# Autodesk Inventor assembly: Escritorio
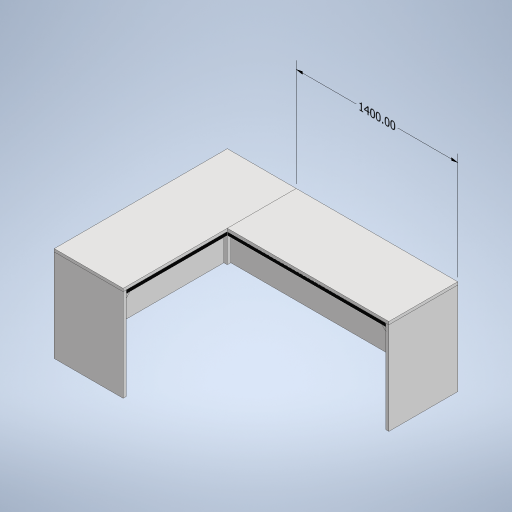
[picture p0: Inventor's stored thumbnail of the model, 512x512]
Saved by Autodesk Inventor 2024 (Build 280153000, 153)
## iProperties
Created: 2023-07-02
Part Number: Escritorio
Document SubType Name: Assembly
Designer: sergi
Author: sergi
## Documents named in this file (17)
- C:\Users\sergi\OneDrive\Escritorio\Piso\Escritorio Piso\Escritorio.iam
- C:\Users\sergi\OneDrive\Escritorio\Piso\Escritorio Piso\Tablero 2.ipt
- C:\Users\sergi\OneDrive\Escritorio\Piso\Escritorio Piso\Lateral1.ipt
- C:\Users\sergi\OneDrive\Escritorio\Piso\Escritorio Piso\Lateral2.ipt
- C:\Users\sergi\OneDrive\Escritorio\Piso\Escritorio Piso\Barra1.ipt
- C:\Users\sergi\OneDrive\Escritorio\Piso\Escritorio Piso\TableroVertical1.ipt
- C:\Users\sergi\OneDrive\Escritorio\Piso\Escritorio Piso\TableroVertical2.ipt
- C:\Users\sergi\OneDrive\Escritorio\Piso\Escritorio Piso\Pata1.ipt
- C:\Users\sergi\OneDrive\Documentos\Tablero Superior Izquierdo.ipt
- C:\Users\sergi\OneDrive\Documentos\Union.ipt
- C:\Users\sergi\OneDrive\Escritorio\Piso\Escritorio Piso\Union.ipt
- C:\Users\sergi\OneDrive\Escritorio\Piso\Escritorio Piso\BarraMarco1.1.ipt
- C:\Users\sergi\OneDrive\Escritorio\Piso\Escritorio Piso\BarraMarco1.2.ipt
- C:\Users\sergi\OneDrive\Escritorio\Piso\Escritorio Piso\BarraMarco2.1.ipt
- C:\Users\sergi\OneDrive\Escritorio\Piso\Escritorio Piso\BarraMarco2.2.ipt
- C:\Users\sergi\OneDrive\Escritorio\Piso\Escritorio Piso\Inclinada3.ipt
- C:\Users\sergi\OneDrive\Escritorio\Piso\Escritorio Piso\Inclinada4.ipt
## Components (26 placed, 15 different names)
1. Tablero 2:1 — Coincidencia:3, Nivelación:5, Nivelación:6, Coincidencia:18, Nivelación:9, Nivelación:14, Coincidencia:52
2. Lateral1:1 — Coincidencia:16, Nivelación:13, Nivelación:15, Coincidencia:20, Nivelación:16, Coincidencia:22, Coincidencia:23, Coincidencia:24, Coincidencia:40, Coincidencia:45
3. Lateral2:1 — Coincidencia:3, Nivelación:5, Nivelación:6, Coincidencia:17, Coincidencia:34, Coincidencia:37, Coincidencia:38, Coincidencia:39, Coincidencia:44
4. Barra1:1 — Coincidencia:19, Nivelación:10, Nivelación:11, Coincidencia:21, Coincidencia:25, Coincidencia:26, Coincidencia:27, Nivelación:17, Coincidencia:35, Nivelación:18, Coincidencia:36
5. TableroVertical1:1 — Coincidencia:16
6. TableroVertical2:1 — Coincidencia:17, Coincidencia:18, Nivelación:9, Nivelación:29, Nivelación:30
7. Pata1:1 — Coincidencia:19, Nivelación:10, Nivelación:11
8. Tablero Superior Izquierdo:1 — Nivelación:13, Nivelación:14, Nivelación:15, Nivelación:17, Coincidencia:41, Nivelación:21, Coincidencia:43, Coincidencia:56, Coincidencia:57, Nivelación:31
9. Union:1 — Coincidencia:20, Coincidencia:21, Nivelación:16, Coincidencia:28
10. Union:2 — Coincidencia:24, Coincidencia:27, Coincidencia:28, Coincidencia:29
11. Union:3 — Coincidencia:23, Coincidencia:26, Coincidencia:29, Coincidencia:30
12. Union:4 — Coincidencia:22, Coincidencia:25, Coincidencia:30, Coincidencia:47
13. Union:5 — Coincidencia:34, Coincidencia:35, Nivelación:18, Nivelación:22
14. Union:6 — Nivelación:19, Coincidencia:37
15. Union:7 — Nivelación:19, Nivelación:20, Coincidencia:38
16. Union:8 — Nivelación:20, Coincidencia:36, Coincidencia:39, Coincidencia:49, Nivelación:23
17. BarraMarco1.1:1 — Coincidencia:40, Coincidencia:41, Nivelación:21, Coincidencia:46
18. BarraMarco1.2:1 — Coincidencia:43, Coincidencia:44, Nivelación:22, Coincidencia:48, Coincidencia:51, Nivelación:24, Nivelación:25
19. BarraMarco2.1:1 — Coincidencia:48, Coincidencia:49, Nivelación:23, Coincidencia:53
20. BarraMarco2.2:1 — Coincidencia:45, Coincidencia:46, Coincidencia:47, Coincidencia:55, Nivelación:27
21. BarraMarco1.2:2 — Nivelación:26, Coincidencia:52, Coincidencia:53
22. BarraMarco2.1:2 — Coincidencia:51, Nivelación:24, Nivelación:25, Nivelación:26
23. BarraMarco1.1:2 — Coincidencia:55, Nivelación:27, Coincidencia:56, Nivelación:28
24. BarraMarco2.2:2 — Nivelación:28, Coincidencia:57
25. Inclinada3:1 — Nivelación:29, Nivelación:30, Nivelación:31, Coincidencia:59, Coincidencia:60
26. Inclinada4:1 — Coincidencia:59, Coincidencia:60
## Relationships (68: Mate 44, Flush 24)
- Coincidencia:3 [Mate]: Tablero 2:1 ↔ Lateral2:1
- Nivelación:5 [Flush]: Tablero 2:1 ↔ Lateral2:1
- Nivelación:6 [Flush]: Tablero 2:1 ↔ Lateral2:1
- Coincidencia:16 [Mate]: Lateral1:1 ↔ TableroVertical1:1
- Coincidencia:17 [Mate]: Lateral2:1 ↔ TableroVertical2:1
- Coincidencia:18 [Mate] (500 mm): Tablero 2:1 ↔ TableroVertical2:1
- Nivelación:9 [Flush]: Tablero 2:1 ↔ TableroVertical2:1
- Coincidencia:19 [Mate]: Barra1:1 ↔ Pata1:1
- Nivelación:10 [Flush]: Barra1:1 ↔ Pata1:1
- Nivelación:11 [Flush]: Barra1:1 ↔ Pata1:1
- Nivelación:13 [Flush]: Lateral1:1 ↔ Tablero Superior Izquierdo:1
- Nivelación:14 [Flush]: Tablero 2:1 ↔ Tablero Superior Izquierdo:1
- Nivelación:15 [Flush]: Lateral1:1 ↔ Tablero Superior Izquierdo:1
- Coincidencia:20 [Mate]: Lateral1:1 ↔ Union:1
- Coincidencia:21 [Mate]: Barra1:1 ↔ Union:1
- Nivelación:16 [Flush]: Lateral1:1 ↔ Union:1
- Coincidencia:22 [Mate]: Lateral1:1 ↔ Union:4
- Coincidencia:23 [Mate]: Lateral1:1 ↔ Union:3
- Coincidencia:24 [Mate]: Lateral1:1 ↔ Union:2
- Coincidencia:25 [Mate]: Barra1:1 ↔ Union:4
- Coincidencia:26 [Mate]: Barra1:1 ↔ Union:3
- Coincidencia:27 [Mate]: Barra1:1 ↔ Union:2
- Coincidencia:28 [Mate] (153.6667 mm): Union:1 ↔ Union:2
- Coincidencia:29 [Mate] (153.667 mm): Union:2 ↔ Union:3
- Coincidencia:30 [Mate] (153.667 mm): Union:3 ↔ Union:4
- Nivelación:17 [Flush]: Barra1:1 ↔ Tablero Superior Izquierdo:1
- [Mate] (153.6667 mm): Union:5 ↔ Union:6
- [Mate] (153.667 mm): Union:6 ↔ Union:7
- [Mate] (153.667 mm): Union:7 ↔ Union:8
- Coincidencia:34 [Mate]: Lateral2:1 ↔ Union:5
- Coincidencia:35 [Mate]: Barra1:1 ↔ Union:5
- Nivelación:18 [Flush]: Barra1:1 ↔ Union:5
- Nivelación:19 [Flush]: Union:6 ↔ Union:7
- Nivelación:20 [Flush]: Union:7 ↔ Union:8
- Coincidencia:36 [Mate]: Barra1:1 ↔ Union:8
- Coincidencia:37 [Mate]: Lateral2:1 ↔ Union:6
- Coincidencia:38 [Mate]: Lateral2:1 ↔ Union:7
- Coincidencia:39 [Mate]: Lateral2:1 ↔ Union:8
- Coincidencia:40 [Mate]: Lateral1:1 ↔ BarraMarco1.1:1
- Coincidencia:41 [Mate]: Tablero Superior Izquierdo:1 ↔ BarraMarco1.1:1
- Nivelación:21 [Flush] (30 mm): Tablero Superior Izquierdo:1 ↔ BarraMarco1.1:1
- Coincidencia:43 [Mate]: Tablero Superior Izquierdo:1 ↔ BarraMarco1.2:1
- Coincidencia:44 [Mate]: Lateral2:1 ↔ BarraMarco1.2:1
- Nivelación:22 [Flush]: Union:5 ↔ BarraMarco1.2:1
- Coincidencia:45 [Mate]: Lateral1:1 ↔ BarraMarco2.2:1
- Coincidencia:46 [Mate]: BarraMarco1.1:1 ↔ BarraMarco2.2:1
- Coincidencia:47 [Mate]: Union:4 ↔ BarraMarco2.2:1
- Coincidencia:48 [Mate]: BarraMarco1.2:1 ↔ BarraMarco2.1:1
- Coincidencia:49 [Mate]: Union:8 ↔ BarraMarco2.1:1
- Nivelación:23 [Flush]: Union:8 ↔ BarraMarco2.1:1
- [Mate]: BarraMarco1.2:2 ↔ BarraMarco2.1:2
- Coincidencia:51 [Mate]: BarraMarco1.2:1 ↔ BarraMarco2.1:2
- Nivelación:24 [Flush]: BarraMarco1.2:1 ↔ BarraMarco2.1:2
- Nivelación:25 [Flush]: BarraMarco1.2:1 ↔ BarraMarco2.1:2
- Nivelación:26 [Flush]: BarraMarco1.2:2 ↔ BarraMarco2.1:2
- Coincidencia:52 [Mate]: Tablero 2:1 ↔ BarraMarco1.2:2
- Coincidencia:53 [Mate]: BarraMarco2.1:1 ↔ BarraMarco1.2:2
- [Mate]: BarraMarco1.1:2 ↔ BarraMarco2.2:2
- Coincidencia:55 [Mate]: BarraMarco2.2:1 ↔ BarraMarco1.1:2
- Nivelación:27 [Flush]: BarraMarco2.2:1 ↔ BarraMarco1.1:2
- Coincidencia:56 [Mate]: Tablero Superior Izquierdo:1 ↔ BarraMarco1.1:2
- Nivelación:28 [Flush]: BarraMarco1.1:2 ↔ BarraMarco2.2:2
- Coincidencia:57 [Mate]: Tablero Superior Izquierdo:1 ↔ BarraMarco2.2:2
- Nivelación:29 [Flush]: TableroVertical2:1 ↔ Inclinada3:1
- Nivelación:30 [Flush]: TableroVertical2:1 ↔ Inclinada3:1
- Nivelación:31 [Flush]: Tablero Superior Izquierdo:1 ↔ Inclinada3:1
- Coincidencia:59 [Mate]: Inclinada3:1 ↔ Inclinada4:1
- Coincidencia:60 [Mate]: Inclinada3:1 ↔ Inclinada4:1
## Named parameters: d55_d51 = 153.66667 mm, d56_d52 = 153.667 mm, d57_d53 = 153.667 mm, d87_d84 = 0 mm, d94_d82 = 0 mm
